# Autodesk Inventor assembly: Test_assembly
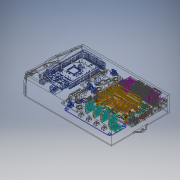
[picture p0: Inventor's stored thumbnail of the model, 180x180]
Saved by Autodesk Inventor 2019 (Build 230136000, 136)
## iProperties
Created: 2020-02-14
Part Number: Test_assembly
Document SubType Name: Assembly
Designer: close
Author: close
## Documents named in this file (6)
- C:\Users\close\Desktop\CAD BARC-ROAR\Enclosure\V_3\Test_assembly_v3.iam
- C:\Users\close\Desktop\CAD BARC-ROAR\Enclosure\V_3\Enclosure_v3.ipt
- C:\Users\close\Desktop\CAD BARC-ROAR\Dependencies\Nvidia Jetson Nano\P3450_P3449_A02_P3448_A02.iam
- C:\Users\close\Desktop\CAD BARC-ROAR\Dependencies\Splitter Board\SplitterBoard.iam
- C:\Users\close\Desktop\CAD BARC-ROAR\Dependencies\Arduino\Mega\arduinoMegaDetailed.ipt
- C:\Users\close\Desktop\CAD BARC-ROAR\Dependencies\Drok Step Down\CN2596-2.iam
## Components (6 placed, 5 different names)
1. Enclosure_v3:1 — Insert:1, Insert:2
2. P3450_P3449_A02_P3448_A02:1 [sub-assembly] — Insert:1, Insert:2
3. SplitterBoard:1 [sub-assembly]
4. arduinoMegaDetailed:1
5. CN2596-2:1 [sub-assembly]
6. CN2596-2:2 [sub-assembly]
## Relationships (2: Insert 2)
- Insert:1: Enclosure_v3:1 ↔ P3450_P3449_A02_P3448_A02:1
- Insert:2: Enclosure_v3:1 ↔ P3450_P3449_A02_P3448_A02:1
